# Autodesk Inventor assembly: Load Cell Hopper Interface_MIR
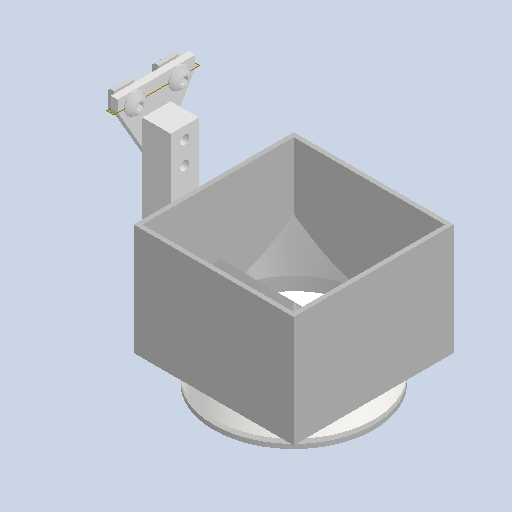
[picture p0: Inventor's stored thumbnail of the model, 512x512]
Saved by Autodesk Inventor 2022 (Build 260153000, 153)
## iProperties
Created: 2022-09-20
Part Number: Load Cell Hopper Interface_MIR
Document SubType Name: Assembly
Designer: Garrett Raker
Author: Garrett Raker
## Documents named in this file (9)
- F:\College Stuff\ATMAE Robotics\Pill Dispenser Robot\Load Cell_Hopper_Connection\Load Cell Hopper Interface_MIR.iam
- F:\College Stuff\ATMAE Robotics\Pill Dispenser Robot\Load Cell_Hopper_Connection\Load_Cell_MIR.ipt
- F:\College Stuff\ATMAE Robotics\Pill Dispenser Robot\Load Cell_Hopper_Connection\Load Cell Connector to Extrusion Bar_MIR.ipt
- F:\College Stuff\ATMAE Robotics\Pill Dispenser Robot\Load Cell_Hopper_Connection\Hopper Connector\Traingular Hopper Connector_MIR.ipt
- F:\College Stuff\ATMAE Robotics\Pill Dispenser Robot\Hoppers\M&M Hopper\M&M Hopper Assembly_MIR.iam
- F:\College Stuff\ATMAE Robotics\Pill Dispenser Robot\Load Cell_Hopper_Connection\T-Nut Block M5  Threads_MIR.ipt
- F:\College Stuff\ATMAE Robotics\Pill Dispenser Robot\Load Cell_Hopper_Connection\M4 25mm Length Flat Head Screw_MIR.ipt
- F:\College Stuff\ATMAE Robotics\Pill Dispenser Robot\Threads and Fasteners\M5 Screw 8mm length_MIR.ipt
- F:\College Stuff\ATMAE Robotics\Pill Dispenser Robot\Base Structure\2811 Series Zinc-Plated Steel Hex Nut (M4 x 0.7mm, 7mm Hex)_MIR1.ipt
## Components (12 placed, 8 different names)
1. Load_Cell_MIR:1 — Mate:34, Mate:33, Mate:7, Mate:10, Mate:9, Mate:8, Mate:23, Mate:24, Mate:31, Mate:32
2. Load Cell Connector to Extrusion Bar_MIR:1 — Mate:34, Mate:33, Mate:7, Mate:15, Mate:20, Mate:14, Mate:19, Mate:27, Mate:25, Mate:28, Mate:26
3. Traingular Hopper Connector_MIR:1 — Mate:10, Mate:9, Mate:8, Mate:13, Mate:12, Mate:11, Flush:1, Flush:2
4. M&M Hopper Assembly_MIR:1 [sub-assembly] — Mate:13, Mate:12, Mate:11
5. T-Nut Block M5  Threads_MIR:1 — Mate:15, Mate:20
6. T-Nut Block M5  Threads_MIR:2 — Mate:14, Mate:19
7. M4 25mm Length Flat Head Screw_MIR:1 — Flush:1, Mate:23, Mate:30
8. M4 25mm Length Flat Head Screw_MIR:2 — Flush:2, Mate:24, Mate:29
9. M5 Screw 8mm length_MIR:1 — Mate:27, Mate:25
10. M5 Screw 8mm length_MIR:2 — Mate:28, Mate:26
11. 2811 Series Zinc-Plated Steel Hex Nut (M4 x 0.7mm, 7mm Hex)_MIR1:1 — Mate:31, Mate:29
12. 2811 Series Zinc-Plated Steel Hex Nut (M4 x 0.7mm, 7mm Hex)_MIR1:2 — Mate:32, Mate:30
## Relationships (25: Mate 22, Flush 3)
- Mate:34: Load_Cell_MIR:1 ↔ Load Cell Connector to Extrusion Bar_MIR:1
- Mate:33: Load_Cell_MIR:1 ↔ Load Cell Connector to Extrusion Bar_MIR:1
- Mate:7: Load_Cell_MIR:1 ↔ Load Cell Connector to Extrusion Bar_MIR:1
- Mate:10: Load_Cell_MIR:1 ↔ Traingular Hopper Connector_MIR:1
- Mate:9: Load_Cell_MIR:1 ↔ Traingular Hopper Connector_MIR:1
- Mate:8: Load_Cell_MIR:1 ↔ Traingular Hopper Connector_MIR:1
- Mate:13: Traingular Hopper Connector_MIR:1 ↔ M&M Hopper Assembly_MIR:1
- Mate:12: Traingular Hopper Connector_MIR:1 ↔ M&M Hopper Assembly_MIR:1
- Mate:11: Traingular Hopper Connector_MIR:1 ↔ M&M Hopper Assembly_MIR:1
- Mate:15: Load Cell Connector to Extrusion Bar_MIR:1 ↔ T-Nut Block M5  Threads_MIR:1
- Mate:20: Load Cell Connector to Extrusion Bar_MIR:1 ↔ T-Nut Block M5  Threads_MIR:1
- Mate:14: Load Cell Connector to Extrusion Bar_MIR:1 ↔ T-Nut Block M5  Threads_MIR:2
- Mate:19 [Flush]: Load Cell Connector to Extrusion Bar_MIR:1 ↔ T-Nut Block M5  Threads_MIR:2
- Flush:1: Traingular Hopper Connector_MIR:1 ↔ M4 25mm Length Flat Head Screw_MIR:1
- Mate:23: Load_Cell_MIR:1 ↔ M4 25mm Length Flat Head Screw_MIR:1
- Flush:2: Traingular Hopper Connector_MIR:1 ↔ M4 25mm Length Flat Head Screw_MIR:2
- Mate:24: Load_Cell_MIR:1 ↔ M4 25mm Length Flat Head Screw_MIR:2
- Mate:27: Load Cell Connector to Extrusion Bar_MIR:1 ↔ M5 Screw 8mm length_MIR:1
- Mate:25: Load Cell Connector to Extrusion Bar_MIR:1 ↔ M5 Screw 8mm length_MIR:1
- Mate:28: Load Cell Connector to Extrusion Bar_MIR:1 ↔ M5 Screw 8mm length_MIR:2
- Mate:26: Load Cell Connector to Extrusion Bar_MIR:1 ↔ M5 Screw 8mm length_MIR:2
- Mate:31: Load_Cell_MIR:1 ↔ 2811 Series Zinc-Plated Steel Hex Nut (M4 x 0.7mm, 7mm Hex)_MIR1:1
- Mate:29: M4 25mm Length Flat Head Screw_MIR:2 ↔ 2811 Series Zinc-Plated Steel Hex Nut (M4 x 0.7mm, 7mm Hex)_MIR1:1
- Mate:32: Load_Cell_MIR:1 ↔ 2811 Series Zinc-Plated Steel Hex Nut (M4 x 0.7mm, 7mm Hex)_MIR1:2
- Mate:30: M4 25mm Length Flat Head Screw_MIR:1 ↔ 2811 Series Zinc-Plated Steel Hex Nut (M4 x 0.7mm, 7mm Hex)_MIR1:2
